# Autodesk Inventor assembly: CNC1
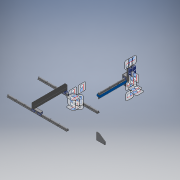
[picture p0: Inventor's stored thumbnail of the model, 180x180]
Saved by Autodesk Inventor 2018 (Build 220112000, 112)
## iProperties
Created: 2018-10-09
Part Number: CNC1
Material: Genérico
Document SubType Name: Assembly
Designer: Georgines
Author: Georgines
## Documents named in this file (12)
- C:\Users\Georgines\Documents\CNC\MONTAGEM\CNC1.iam
- C:\Users\Georgines\Documents\CNC\COMPONENTES_MECANICOS\GUIAS_LINEARES\SBR16.ipt
- C:\Users\Georgines\Documents\CNC\COMPONENTES_MECANICOS\BLOCOS_GUIAS_LINEARES\SBR16UU.ipt
- C:\Users\Georgines\Documents\CNC\COMPONENTES_MECANICOS\PERFIL_ESTRUTURAL\PERFIL_ESTRUTURAL_40X80_585MM.ipt
- C:\Users\Georgines\Documents\CNC\MONTAGEM\CNC1\APOIO_PERFIL_STRUTURAL.ipt
- C:\Users\Georgines\Documents\CNC\MONTAGEM\CNC1\LATERAL_BLOCOS_BASE.ipt
- C:\Users\Georgines\Documents\CNC\MONTAGEM\CNC1\EIXOS_X_Z.iam
- C:\Users\Georgines\Documents\CNC\COMPONENTES_MECANICOS\GUIAS_LINEARES\SBR16_COMPLEMENTENTO.ipt
- C:\Users\Georgines\Documents\CNC\COMPONENTES_MECANICOS\PERFIL_ESTRUTURAL\PERFIL_ESTRUTURAL_30X60_640MM.ipt
- C:\Users\Georgines\Documents\CNC\MONTAGEM\BARRA_SUP_INF_EIXO_X.ipt
- C:\Users\Georgines\Documents\CNC\MONTAGEM\BLOCO_SUPORTE_EIXO_Z.ipt
- C:\Users\Georgines\Documents\CNC\MONTAGEM\CNC1\BLOCO_SUPORTE_EIXO_Z_TRASEIRO.ipt
## Components (41 placed, 11 different names)
1. SBR16:1 — Coincidência:6, Alinhamento:11, Alinhamento:12, Coincidência:13, PARALELO_GUIAS_BASE, DISTANCIA_GUIAS_BASE, ENCAIXE_GUIA_BASE, ENCAIXE_GUIA_BASE_2
2. SBR16:2 — Alinhamento:9, Coincidência:5, Alinhamento:10, Coincidência:6, Alinhamento:11, Alinhamento:12
3. SBR16:3 — Coincidência:4, Alinhamento:4, Alinhamento:8, Alinhamento:9, Coincidência:5, Alinhamento:10
4. SBR16:4 — Coincidência:3, Alinhamento:3, Coincidência:4, Alinhamento:4, Alinhamento:7, Alinhamento:8
5. SBR16:5 — Coincidência:2, Alinhamento:2, Coincidência:3, Alinhamento:3, Alinhamento:6, Alinhamento:7
6. SBR16:6 — Coincidência:1, Alinhamento:1, Coincidência:2, Alinhamento:2, Alinhamento:5, Alinhamento:6
7. SBR16:7 — Coincidência:1, Alinhamento:1, Alinhamento:5
8. SBR16:8 — PARALELO_GUIAS_BASE, DISTANCIA_GUIAS_BASE, ENCAIXE_GUIA_BASE_3, ENCAIXE_GUIA_BASE_4
9. SBR16:9 — Coincidência:14
10. SBR16:10
11. SBR16:11
12. SBR16:12
13. SBR16:13
14. SBR16:14
15. SBR16UU:1 — ENCAIXE_GUIA_BASE, ALINHAMENTO_BOCOS_BASE, ALINHAMENTO_BOCOS_BASE_4, ALINHAMENTO_BOCOS_BASE_6, Coincidência:20, Alinhamento:32, Alinhamento:33, Coincidência:22
16. SBR16UU:2 — ENCAIXE_GUIA_BASE_2, ALINHAMENTO_BOCOS_BASE_2, ALINHAMENTO_BOCOS_BASE_4, ALINHAMENTO_BOCOS_BASE_5, Coincidência:20, Alinhamento:31
17. SBR16UU:3 — ENCAIXE_GUIA_BASE_4, ALINHAMENTO_BOCOS_BASE_2, ALINHAMENTO_BOCOS_BASE_5
18. SBR16UU:4 — ENCAIXE_GUIA_BASE_3, ALINHAMENTO_BOCOS_BASE, ALINHAMENTO_BOCOS_BASE_6
19. PERFIL_ESTRUTURAL_40X80_585MM:1 — Coincidência:21, Alinhamento:34, Alinhamento:35
20. APOIO_PERFIL_STRUTURAL:1 — Alinhamento:31, Coincidência:21, Alinhamento:32, Alinhamento:33, Coincidência:22, Alinhamento:34, Alinhamento:35, Alinhamento:36
21. LATERAL_BLOCOS_BASE:1 — Alinhamento:36
22. EIXOS_X_Z:1 [sub-assembly] — Coincidência:44, Coincidência:47, Alinhamento:77, Alinhamento:78
23. SBR16:15
24. SBR16:16
25. SBR16:17
26. SBR16:18 — Coincidência:30, Alinhamento:49, Alinhamento:50, Coincidência:31, Coincidência:39, Coincidência:40
27. SBR16_COMPLEMENTENTO:1 — Coincidência:30, Alinhamento:49, Alinhamento:50, Alinhamento:51, Alinhamento:52
28. PERFIL_ESTRUTURAL_30X60_640MM:1 — Coincidência:31, Alinhamento:51, Alinhamento:52, Coincidência:36, Alinhamento:61, Alinhamento:62
29. SBR16:19 — Alinhamento:61, Alinhamento:62, Coincidência:37, Coincidência:38
30. SBR16:20
31. SBR16:21
32. SBR16:22 — Coincidência:36
33. SBR16_COMPLEMENTENTO:2
34. SBR16UU:5 — Coincidência:39, Alinhamento:63, Alinhamento:65, Coincidência:41, Coincidência:42, Alinhamento:67
35. SBR16UU:6 — Coincidência:40, Alinhamento:64, Alinhamento:66, Coincidência:41, Alinhamento:68
36. SBR16UU:7 — Coincidência:37, Alinhamento:63, Alinhamento:65, Alinhamento:69
37. SBR16UU:8 — Coincidência:38, Alinhamento:64, Alinhamento:66, Coincidência:43
38. BARRA_SUP_INF_EIXO_X:1 — Coincidência:42, Alinhamento:67, Alinhamento:68, Alinhamento:70, Alinhamento:71, Alinhamento:72, Coincidência:45, Alinhamento:73, Coincidência:46, Alinhamento:76
39. BARRA_SUP_INF_EIXO_X:2 — Coincidência:43, Alinhamento:69, Alinhamento:70, Alinhamento:74, Alinhamento:75
40. BLOCO_SUPORTE_EIXO_Z:1 — Alinhamento:71, Coincidência:44, Coincidência:45, Alinhamento:73, Alinhamento:74, Coincidência:47, Alinhamento:77, Alinhamento:78
41. BLOCO_SUPORTE_EIXO_Z_TRASEIRO:1 — Alinhamento:72, Alinhamento:75, Coincidência:46, Alinhamento:76
## Relationships (115: Flush 72, Mate 43)
- Coincidência:1 [Mate]: SBR16:6 ↔ SBR16:7
- Alinhamento:1 [Flush]: SBR16:6 ↔ SBR16:7
- Coincidência:2 [Mate]: SBR16:5 ↔ SBR16:6
- Alinhamento:2 [Flush]: SBR16:5 ↔ SBR16:6
- Coincidência:3 [Mate]: SBR16:4 ↔ SBR16:5
- Alinhamento:3 [Flush]: SBR16:4 ↔ SBR16:5
- Coincidência:4 [Mate]: SBR16:3 ↔ SBR16:4
- Alinhamento:4 [Flush]: SBR16:3 ↔ SBR16:4
- Alinhamento:5 [Flush]: SBR16:6 ↔ SBR16:7
- Alinhamento:6 [Flush]: SBR16:5 ↔ SBR16:6
- Alinhamento:7 [Flush]: SBR16:4 ↔ SBR16:5
- Alinhamento:8 [Flush]: SBR16:3 ↔ SBR16:4
- Alinhamento:9 [Flush]: SBR16:2 ↔ SBR16:3
- Coincidência:5 [Mate]: SBR16:2 ↔ SBR16:3
- Alinhamento:10 [Flush]: SBR16:2 ↔ SBR16:3
- Coincidência:6 [Mate]: SBR16:1 ↔ SBR16:2
- Alinhamento:11 [Flush]: SBR16:1 ↔ SBR16:2
- Alinhamento:12 [Flush]: SBR16:1 ↔ SBR16:2
- [Mate]: SBR16:13 ↔ SBR16:14
- [Flush]: SBR16:13 ↔ SBR16:14
- [Mate]: SBR16:12 ↔ SBR16:13
- [Flush]: SBR16:12 ↔ SBR16:13
- [Mate]: SBR16:11 ↔ SBR16:12
- [Flush]: SBR16:11 ↔ SBR16:12
- [Mate]: SBR16:10 ↔ SBR16:11
- [Flush]: SBR16:10 ↔ SBR16:11
- [Flush]: SBR16:13 ↔ SBR16:14
- [Flush]: SBR16:12 ↔ SBR16:13
- [Flush]: SBR16:11 ↔ SBR16:12
- [Flush]: SBR16:10 ↔ SBR16:11
- [Flush]: SBR16:9 ↔ SBR16:10
- [Mate]: SBR16:9 ↔ SBR16:10
- [Flush]: SBR16:9 ↔ SBR16:10
- [Mate]: SBR16:8 ↔ SBR16:9
- [Flush]: SBR16:8 ↔ SBR16:9
- [Flush]: SBR16:8 ↔ SBR16:9
- Coincidência:13 [Mate]: SBR16:1
- Coincidência:14 [Mate]: SBR16:9
- PARALELO_GUIAS_BASE [Flush]: SBR16:1 ↔ SBR16:8
- DISTANCIA_GUIAS_BASE [Mate] (500 mm): SBR16:1 ↔ SBR16:8
- ENCAIXE_GUIA_BASE [Mate]: SBR16:1 ↔ SBR16UU:1
- ENCAIXE_GUIA_BASE_2 [Mate]: SBR16:1 ↔ SBR16UU:2
- ENCAIXE_GUIA_BASE_3 [Mate]: SBR16:8 ↔ SBR16UU:4
- ENCAIXE_GUIA_BASE_4 [Mate]: SBR16:8 ↔ SBR16UU:3
- ALINHAMENTO_BOCOS_BASE [Flush]: SBR16UU:1 ↔ SBR16UU:4
- ALINHAMENTO_BOCOS_BASE_2 [Flush]: SBR16UU:2 ↔ SBR16UU:3
- ALINHAMENTO_BOCOS_BASE_4 [Flush]: SBR16UU:1 ↔ SBR16UU:2
- ALINHAMENTO_BOCOS_BASE_5 [Flush]: SBR16UU:2 ↔ SBR16UU:3
- ALINHAMENTO_BOCOS_BASE_6 [Flush]: SBR16UU:1 ↔ SBR16UU:4
- Coincidência:20 [Mate] (60 mm): SBR16UU:1 ↔ SBR16UU:2
- Alinhamento:31 [Flush]: SBR16UU:2 ↔ APOIO_PERFIL_STRUTURAL:1
- Coincidência:21 [Mate]: PERFIL_ESTRUTURAL_40X80_585MM:1 ↔ APOIO_PERFIL_STRUTURAL:1
- Alinhamento:32 [Flush]: SBR16UU:1 ↔ APOIO_PERFIL_STRUTURAL:1
- Alinhamento:33 [Flush]: SBR16UU:1 ↔ APOIO_PERFIL_STRUTURAL:1
- Coincidência:22 [Mate]: SBR16UU:1 ↔ APOIO_PERFIL_STRUTURAL:1
- Alinhamento:34 [Flush]: PERFIL_ESTRUTURAL_40X80_585MM:1 ↔ APOIO_PERFIL_STRUTURAL:1
- Alinhamento:35 [Flush] (-110 mm): PERFIL_ESTRUTURAL_40X80_585MM:1 ↔ APOIO_PERFIL_STRUTURAL:1
- Alinhamento:36 [Flush]: APOIO_PERFIL_STRUTURAL:1 ↔ LATERAL_BLOCOS_BASE:1
- [Mate]: SBR16:17 ↔ SBR16:18
- [Flush]: SBR16:17 ↔ SBR16:18
- [Flush]: SBR16:17 ↔ SBR16:18
- [Flush]: SBR16:16 ↔ SBR16:17
- [Mate]: SBR16:16 ↔ SBR16:17
- [Flush]: SBR16:16 ↔ SBR16:17
- [Mate]: SBR16:15 ↔ SBR16:16
- [Flush]: SBR16:15 ↔ SBR16:16
- [Flush]: SBR16:15 ↔ SBR16:16
- Coincidência:30 [Mate]: SBR16:18 ↔ SBR16_COMPLEMENTENTO:1
- Alinhamento:49 [Flush]: SBR16:18 ↔ SBR16_COMPLEMENTENTO:1
- Alinhamento:50 [Flush]: SBR16:18 ↔ SBR16_COMPLEMENTENTO:1
- Coincidência:31 [Mate]: SBR16:18 ↔ PERFIL_ESTRUTURAL_30X60_640MM:1
- Alinhamento:51 [Flush]: SBR16_COMPLEMENTENTO:1 ↔ PERFIL_ESTRUTURAL_30X60_640MM:1
- Alinhamento:52 [Flush] (10 mm): SBR16_COMPLEMENTENTO:1 ↔ PERFIL_ESTRUTURAL_30X60_640MM:1
- [Mate]: SBR16:21 ↔ SBR16:22
- [Flush]: SBR16:21 ↔ SBR16:22
- [Flush]: SBR16:21 ↔ SBR16:22
- [Flush]: SBR16:20 ↔ SBR16:21
- [Mate]: SBR16:20 ↔ SBR16:21
- [Flush]: SBR16:20 ↔ SBR16:21
- [Mate]: SBR16:19 ↔ SBR16:20
- [Flush]: SBR16:19 ↔ SBR16:20
- [Flush]: SBR16:19 ↔ SBR16:20
- [Mate]: SBR16:22 ↔ SBR16_COMPLEMENTENTO:2
- [Flush]: SBR16:22 ↔ SBR16_COMPLEMENTENTO:2
- [Flush]: SBR16:22 ↔ SBR16_COMPLEMENTENTO:2
- Coincidência:36 [Mate]: PERFIL_ESTRUTURAL_30X60_640MM:1 ↔ SBR16:22
- Alinhamento:61 [Flush]: PERFIL_ESTRUTURAL_30X60_640MM:1 ↔ SBR16:19
- Alinhamento:62 [Flush] (-10 mm): PERFIL_ESTRUTURAL_30X60_640MM:1 ↔ SBR16:19
- Coincidência:37 [Mate]: SBR16:19 ↔ SBR16UU:7
- Coincidência:38 [Mate]: SBR16:19 ↔ SBR16UU:8
- Coincidência:39 [Mate]: SBR16:18 ↔ SBR16UU:5
- Coincidência:40 [Mate]: SBR16:18 ↔ SBR16UU:6
- Alinhamento:63 [Flush]: SBR16UU:5 ↔ SBR16UU:7
- Alinhamento:64 [Flush]: SBR16UU:6 ↔ SBR16UU:8
- Alinhamento:65 [Flush]: SBR16UU:5 ↔ SBR16UU:7
- Alinhamento:66 [Flush]: SBR16UU:6 ↔ SBR16UU:8
- Coincidência:41 [Mate] (15 mm): SBR16UU:5 ↔ SBR16UU:6
- Coincidência:42 [Mate]: SBR16UU:5 ↔ BARRA_SUP_INF_EIXO_X:1
- Alinhamento:67 [Flush] (12.5 mm): SBR16UU:5 ↔ BARRA_SUP_INF_EIXO_X:1
- Alinhamento:68 [Flush]: SBR16UU:6 ↔ BARRA_SUP_INF_EIXO_X:1
- Coincidência:43 [Mate]: SBR16UU:8 ↔ BARRA_SUP_INF_EIXO_X:2
- Alinhamento:69 [Flush]: SBR16UU:7 ↔ BARRA_SUP_INF_EIXO_X:2
- Alinhamento:70 [Flush]: BARRA_SUP_INF_EIXO_X:1 ↔ BARRA_SUP_INF_EIXO_X:2
- Alinhamento:71 [Flush]: BARRA_SUP_INF_EIXO_X:1 ↔ BLOCO_SUPORTE_EIXO_Z:1
- Alinhamento:72 [Flush]: BARRA_SUP_INF_EIXO_X:1 ↔ BLOCO_SUPORTE_EIXO_Z_TRASEIRO:1
- Coincidência:44 [Mate]: EIXOS_X_Z:1 ↔ BLOCO_SUPORTE_EIXO_Z:1
- Coincidência:45 [Mate]: BARRA_SUP_INF_EIXO_X:1 ↔ BLOCO_SUPORTE_EIXO_Z:1
- Alinhamento:73 [Flush]: BARRA_SUP_INF_EIXO_X:1 ↔ BLOCO_SUPORTE_EIXO_Z:1
- Alinhamento:74 [Flush]: BARRA_SUP_INF_EIXO_X:2 ↔ BLOCO_SUPORTE_EIXO_Z:1
- Alinhamento:75 [Flush]: BARRA_SUP_INF_EIXO_X:2 ↔ BLOCO_SUPORTE_EIXO_Z_TRASEIRO:1
- Coincidência:46 [Mate]: BARRA_SUP_INF_EIXO_X:1 ↔ BLOCO_SUPORTE_EIXO_Z_TRASEIRO:1
- Alinhamento:76 [Flush]: BARRA_SUP_INF_EIXO_X:1 ↔ BLOCO_SUPORTE_EIXO_Z_TRASEIRO:1
- Coincidência:47 [Mate]: EIXOS_X_Z:1 ↔ BLOCO_SUPORTE_EIXO_Z:1
- Alinhamento:77 [Flush]: EIXOS_X_Z:1 ↔ BLOCO_SUPORTE_EIXO_Z:1
- Alinhamento:78 [Flush]: EIXOS_X_Z:1 ↔ BLOCO_SUPORTE_EIXO_Z:1
## Named parameters: d23_d20 = 0 mm, d24_d21 = 0 mm, d25_d22 = 0 mm, d26_d5 = 0 mm, d27_d6 = 0 mm, d28_d7 = 0 mm, d29_d8 = 0 mm, d30_d9 = 0 mm, d31_d10 = 0 mm, d32_d11 = 0 mm, d33_d12 = 0 mm, d34_d13 = 0 mm, d35_d14 = 0 mm, d36_d15 = 0 mm, d37_d16 = 0 mm, d38_d17 = 0 mm, d39_d18 = 0 mm, d40_d19 = 0 mm, d65_d23_d20 = 0 mm, d66_d24_d21 = 0 mm, d67_d25_d22 = 0 mm, d74_d32_d11 = 0 mm, d75_d33_d12 = 0 mm, d79_d37_d16 = 0 mm, d80_d38_d17 = 0 mm, d81_d39_d18 = 0 mm, d82_d40_d19 = 0 mm, d91_d85 = 0 mm, d92_d86 = 0 mm, d93_d87 = 0 mm, d94_d65_d23_d20 = 0 mm, d95_d66_d24_d21 = 0 mm, d96_d67_d25_d22 = 0 mm, d97_d74_d32_d11 = 0 mm, d98_d75_d33_d12 = 0 mm, d99_d79_d37_d16 = 0 mm, d100_d80_d38_d17 = 0 mm, d101_d81_d39_d18 = 0 mm, d102_d82_d40_d19 = 0 mm
